# Autodesk Inventor assembly: Montagem
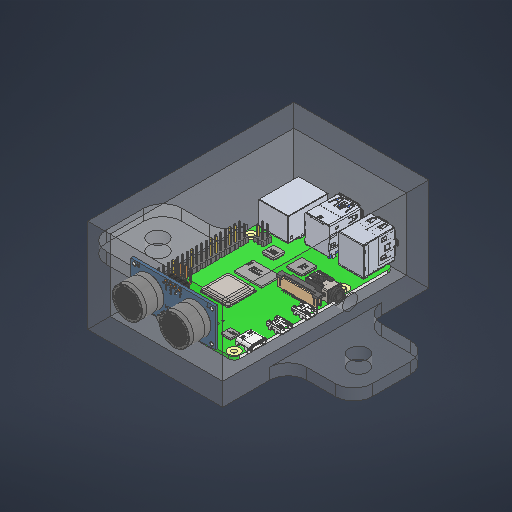
[picture p0: Inventor's stored thumbnail of the model, 512x512]
Saved by Autodesk Inventor 2026 (Build 300175050, 175E)
## iProperties
Created: 2025-09-06
Part Number: Montagem
Document SubType Name: Assembly
Designer: alanl
Author: alanl
## Documents named in this file (4)
- C:\Users\alanl\OneDrive\Documentos\Inventor\Hydrowatch\Montagem.iam
- C:\Users\alanl\OneDrive\Documentos\Inventor\Hydrowatch\hc-sr04.ipt
- C:\Users\alanl\OneDrive\Documentos\Inventor\Hydrowatch\Raspberry Pi 4 Model B.ipt
- C:\Users\alanl\OneDrive\Documentos\Inventor\Hydrowatch\Prototipo.ipt
## Components (3 placed, 3 different names)
1. hc-sr04:1 — Rígida:1
2. Raspberry Pi 4 Model B:1 — Coincidente:1, Coincidente:2, Coincidente:3
3. Prototipo:1 — Coincidente:1, Rígida:1, Coincidente:2, Coincidente:3
## Relationships (4: Mate 3, WeldJoint 1)
- Coincidente:1 [Mate] (4 mm): Raspberry Pi 4 Model B:1 ↔ Prototipo:1
- Rígida:1 [WeldJoint] (-3.1 mm): hc-sr04:1 ↔ Prototipo:1
- Coincidente:2 [Mate] (2 mm): Raspberry Pi 4 Model B:1 ↔ Prototipo:1
- Coincidente:3 [Mate]: Raspberry Pi 4 Model B:1 ↔ Prototipo:1
